# Autodesk Inventor assembly: CimMotorAnd4inWheel
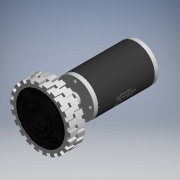
[picture p0: Inventor's stored thumbnail of the model, 180x180]
Saved by Autodesk Inventor 2016 SP1 (Build 200210100, 210)
## iProperties
Created: 2016-01-21
Part Number: CimMotorAnd4inWheel
Document SubType Name: Assembly
Designer: steele
Author: steele
## Documents named in this file (3)
- C:\snobotics\CAD-Development\robSteele\SnoBotics2016\2ndCutAtPitchingMachineRobot\CimMotorAnd4inWheel.iam
- C:\snobotics\autodesk\2015\FRC_KOP_2015\Motors\MOT_CIM-Motor_217-2000.iam
- C:\snobotics\autodesk\2015\FRC_KOP_2015\Drive Base\Parts\4 in HiGrip Wheel.iam
## Components (2 placed, 2 different names)
1. MOT_CIM-Motor_217-2000:1 [sub-assembly] — Insert:1
2. 4 in HiGrip Wheel:1 [sub-assembly] — Insert:1
## Relationships (1: Insert 1)
- Insert:1: MOT_CIM-Motor_217-2000:1 ↔ 4 in HiGrip Wheel:1
